# Autodesk Inventor assembly: FullLegAssembly
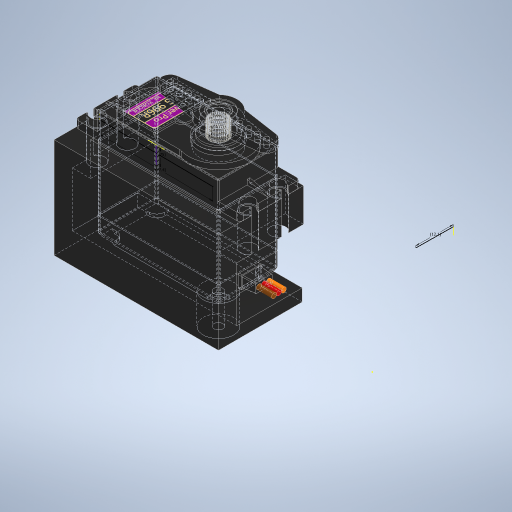
[picture p0: Inventor's stored thumbnail of the model, 512x512]
Saved by Autodesk Inventor 2024 (Build 280153000, 153)
## iProperties
Created: 2024-09-10
Part Number: FullLegAssembly
Document SubType Name: Assembly
Designer: omiye
Author: omiye
## Documents named in this file (4)
- C:\Projects\Arduino\hexapod\legModels\FullLegAssembly.iam
- C:\Projects\Arduino\hexapod\legModels\MG996RServo.ipt
- C:\Projects\Arduino\hexapod\legModels\MG996RServoHolder.ipt
- C:\Projects\Arduino\hexapod\legModels\straightServoHorn.ipt
## Components (3 placed, 3 different names)
1. MG996RServo:1 — Mate:1, Mate:2, Mate:3, Mate:4, Mate:5, Mate:6
2. MG996RServoHolder:1 — Mate:1, Mate:2, Mate:3, Mate:4
3. straightServoHorn:1 — Mate:5, Mate:6
## Relationships (6: Mate 6)
- Mate:1: MG996RServo:1 ↔ MG996RServoHolder:1
- Mate:2: MG996RServo:1 ↔ MG996RServoHolder:1
- Mate:3: MG996RServo:1 ↔ MG996RServoHolder:1
- Mate:4: MG996RServo:1 ↔ MG996RServoHolder:1
- Mate:5: MG996RServo:1 ↔ straightServoHorn:1
- Mate:6: MG996RServo:1 ↔ straightServoHorn:1
